# Autodesk Inventor assembly: beanIntake-v2
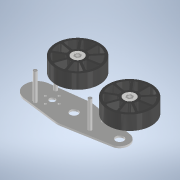
[picture p0: Inventor's stored thumbnail of the model, 180x180]
Saved by Autodesk Inventor 2020 (Build 240168000, 168)
## iProperties
Created: 2020-01-04
Part Number: beanIntake-v2
Document SubType Name: Assembly
Designer: xj82b
Author: xj82b
## Documents named in this file (5)
- C:\Users\xj82b\Documents\Inventor\5199\beanIntake-v2.iam
- C:\Users\xj82b\Documents\Inventor\5199\bottombeanv2.ipt
- C:\Users\xj82b\Documents\Inventor\5199\gobilda parts\1501-0006-0480.ipt
- C:\Users\xj82b\Documents\Inventor\5199\andymark parts\am-3946 3IN 375Hex Compliant Wheel VER 3.ipt
- C:\Users\xj82b\Documents\Inventor\5199\5mm.125in insert.ipt
## Components (9 placed, 4 different names)
1. bottombeanv2:1 — Mate:1, Mate:2, Mate:3, Mate:4, Mate:5, Mate:6, Mate:7, Mate:8
2. 1501-0006-0480:1 — Mate:1, Mate:6
3. 1501-0006-0480:2 — Mate:2, Mate:8
4. 1501-0006-0480:3 — Mate:3, Mate:7
5. 1501-0006-0480:4 — Mate:4, Mate:5
6. am-3946 3IN 375Hex Compliant Wheel VER 3:1 — Mate:9, Mate:10, Mate:11
7. am-3946 3IN 375Hex Compliant Wheel VER 3:2 — Mate:12, Mate:13, Mate:14
8. 5mm.125in insert:1 — Mate:9, Mate:10, Mate:11
9. 5mm.125in insert:2 — Mate:12, Mate:13, Mate:14
## Relationships (14: Mate 14)
- Mate:1: bottombeanv2:1 ↔ 1501-0006-0480:1
- Mate:2: bottombeanv2:1 ↔ 1501-0006-0480:2
- Mate:3: bottombeanv2:1 ↔ 1501-0006-0480:3
- Mate:4: bottombeanv2:1 ↔ 1501-0006-0480:4
- Mate:5: bottombeanv2:1 ↔ 1501-0006-0480:4
- Mate:6: bottombeanv2:1 ↔ 1501-0006-0480:1
- Mate:7: bottombeanv2:1 ↔ 1501-0006-0480:3
- Mate:8: bottombeanv2:1 ↔ 1501-0006-0480:2
- Mate:9: am-3946 3IN 375Hex Compliant Wheel VER 3:1 ↔ 5mm.125in insert:1
- Mate:10: am-3946 3IN 375Hex Compliant Wheel VER 3:1 ↔ 5mm.125in insert:1
- Mate:11: am-3946 3IN 375Hex Compliant Wheel VER 3:1 ↔ 5mm.125in insert:1
- Mate:12: am-3946 3IN 375Hex Compliant Wheel VER 3:2 ↔ 5mm.125in insert:2
- Mate:13: am-3946 3IN 375Hex Compliant Wheel VER 3:2 ↔ 5mm.125in insert:2
- Mate:14: am-3946 3IN 375Hex Compliant Wheel VER 3:2 ↔ 5mm.125in insert:2
